# Autodesk Inventor assembly: Reward spout
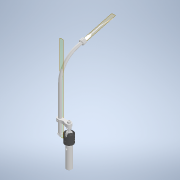
[picture p0: Inventor's stored thumbnail of the model, 180x180]
Saved by Autodesk Inventor 2021.2 (Build 252289000, 289)
## iProperties
Created: 2021-07-06
Part Number: Reward spout
Document SubType Name: Assembly
Designer: jl4459
Author: jl4459
## Documents named in this file (9)
- C:\Users\jl4459\Documents\Inventor\Training mini VR rig\Modules\Reward\Reward spout.iam
- C:\Users\jl4459\Documents\Inventor\Training mini VR rig\Modules\Reward\Parts\Stainless steel tube.ipt
- C:\Users\jl4459\Documents\Inventor\Training mini VR rig\Modules\Reward\Parts\51525K428_PLASTIC QUICK-TURN TUBE COUPLING.ipt
- C:\Users\jl4459\Documents\Inventor\Training mini VR rig\Modules\Reward\Parts\4406T110_MINIATURE STAINLESS STEEL BARBED TUBE FITTING.ipt
- C:\Users\jl4459\Documents\Inventor\Training mini VR rig\Modules\Reward\Parts\Syringe Needle, With Luer - White-17Gauge.ipt
- C:\Users\jl4459\Documents\Inventor\Training mini VR rig\Modules\Reward\Parts\Tube to TRB1 adapter.ipt
- C:\Users\jl4459\Documents\Inventor\Training mini VR rig\Modules\Reward\Parts\TRB1-Step.ipt
- C:\Users\jl4459\Documents\Inventor\Training mini VR rig\Modules\Reward\Parts\91251A194_Black-Oxide Alloy Steel Socket Head Screw.ipt
- C:\Users\jl4459\Documents\Inventor\Training mini VR rig\Modules\Reward\Parts\TR2-Step(1).ipt
## Components (8 placed, 8 different names)
1. Stainless steel tube:1
2. 51525K428_PLASTIC QUICK-TURN TUBE COUPLING:1
3. 4406T110_MINIATURE STAINLESS STEEL BARBED TUBE FITTING:1
4. Syringe Needle, With Luer - White-17Gauge:1
5. Tube to TRB1 adapter:1
6. TRB1-Step:1
7. 91251A194_Black-Oxide Alloy Steel Socket Head Screw:1
8. TR2-Step(1):1
## Relationships (7: Insert 7)
- [Insert] (-6.35 mm): Stainless steel tube:1 ↔ 4406T110_MINIATURE STAINLESS STEEL BARBED TUBE FITTING:1
- [Insert] (-5.08 mm): 51525K428_PLASTIC QUICK-TURN TUBE COUPLING:1 ↔ Syringe Needle, With Luer - White-17Gauge:1
- [Insert] (-6.35 mm): Stainless steel tube:1 ↔ 51525K428_PLASTIC QUICK-TURN TUBE COUPLING:1
- [Insert] (-76.2 mm): Stainless steel tube:1 ↔ Tube to TRB1 adapter:1
- [Insert]: Tube to TRB1 adapter:1 ↔ 91251A194_Black-Oxide Alloy Steel Socket Head Screw:1
- [Insert] (-6.35 mm): TRB1-Step:1 ↔ 91251A194_Black-Oxide Alloy Steel Socket Head Screw:1
- [Insert] (-4.064 mm): TRB1-Step:1 ↔ TR2-Step(1):1
